# Autodesk Inventor assembly: Heatpipe
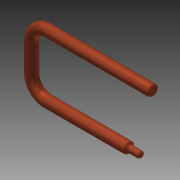
[picture p0: Inventor's stored thumbnail of the model, 180x180]
Saved by Autodesk Inventor 2015 (Build 190159000, 159)
## iProperties
Created: 2015-08-22
Part Number: Heatpipe
Document SubType Name: Assembly
Designer: Kyle
Author: Kyle
## Documents named in this file (3)
- C:\Users\Kyle\Documents\Project documentation\Supermicro X7DCA-L Watercooling\Heatpipe.iam
- C:\Users\Kyle\Documents\Project documentation\Supermicro X7DCA-L Watercooling\Copper_tube.ipt
- C:\Users\Kyle\Documents\Project documentation\Supermicro X7DCA-L Watercooling\Water_tube.ipt
## Components (2 placed, 2 different names)
1. Copper_tube:1 — Mate:1, Mate:2, Mate:3
2. Water_tube:1 — Mate:1, Mate:2, Mate:3
## Relationships (3: Mate 3)
- Mate:1: Copper_tube:1 ↔ Water_tube:1
- Mate:2: Copper_tube:1 ↔ Water_tube:1
- Mate:3: Copper_tube:1 ↔ Water_tube:1
